# Autodesk Inventor assembly: riasedMarkerWithKey
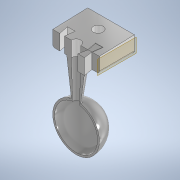
[picture p0: Inventor's stored thumbnail of the model, 180x180]
Saved by Autodesk Inventor 2022 (Build 260153000, 153)
## iProperties
Created: 2021-09-22
Part Number: riasedMarkerWithKey
Document SubType Name: Assembly
Designer: tecware
Author: tecware
## Documents named in this file (3)
- C:\Users\tecware\Documents\git\calibrationKit\L-frame\components_L-frame\riasedMarkerWithKey.iam
- C:\Users\tecware\Documents\git\calibrationKit\L-frame\components_L-frame\raisedMarkerWIthBase.ipt
- C:\Users\tecware\Documents\git\calibrationKit\L-frame\components_L-frame\raisedMarkerWIthBase-key.ipt
## Components (2 placed, 2 different names)
1. raisedMarkerWIthBase:1 — Flush:1
2. raisedMarkerWIthBase-key:1 — Flush:1
## Relationships (1: Flush 1)
- Flush:1: raisedMarkerWIthBase:1 ↔ raisedMarkerWIthBase-key:1
